# Autodesk Inventor assembly: Draft_02_Combined
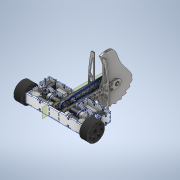
[picture p0: Inventor's stored thumbnail of the model, 180x180]
Saved by Autodesk Inventor 2022 (Build 260153000, 153)
## iProperties
Created: 2021-03-10
Part Number: Draft_02_Combined
Document SubType Name: Assembly
Designer: M3rob
Mass: 100397 g
Surface Area: 45638.5 cm^2
Volume: 29165.9 cm^3
Density: 3.44228 g/cm^3
Author: M3rob
## Documents named in this file (33)
- C:\Users\M3rob\Documents\GrabCAD\FireBird 250 Pound Gaming Machine\Drafts\FrameDrafts\Draft_03\Draft_03_Combined.iam
- C:\Users\M3rob\Documents\GrabCAD\FireBird 250 Pound Gaming Machine\Drafts\FrameDrafts\Draft_03\NeckFrame_03.ipt
- C:\Users\M3rob\Documents\GrabCAD\FireBird 250 Pound Gaming Machine\Drafts\FrameDrafts\Draft_03\FrontWallFrame_03.ipt
- C:\Users\M3rob\Documents\GrabCAD\FireBird 250 Pound Gaming Machine\Drafts\FrameDrafts\Draft_03\BackWallFrame_03.ipt
- C:\Users\M3rob\Documents\GrabCAD\FireBird 250 Pound Gaming Machine\Drafts\FrameDrafts\Draft_03\SmallSideFrame_03.ipt
- C:\Users\M3rob\Documents\GrabCAD\FireBird 250 Pound Gaming Machine\Drafts\FrameDrafts\Draft_03\DriveSideFrame_03.ipt
- C:\Users\M3rob\Documents\GrabCAD\FireBird 250 Pound Gaming Machine\Drafts\FrameDrafts\Draft_03\6524K421_FRICTION TORQUE LIMITER.ipt
- C:\Users\M3rob\Documents\GrabCAD\FireBird 250 Pound Gaming Machine\Drafts\FrameDrafts\Draft_03\MotorMountingPlates.ipt
- C:\Users\M3rob\Documents\GrabCAD\FireBird 250 Pound Gaming Machine\Drafts\FrameDrafts\Draft_03\MotorMockup.ipt
- C:\Users\M3rob\Documents\GrabCAD\FireBird 250 Pound Gaming Machine\Drafts\FrameDrafts\Draft_03\GearboxMockup.ipt
- C:\Users\M3rob\Documents\Inventor\Content Center Files\R2021\en-US\AS 2465(2)\AS 2465 - 3_8 x 1 1_4  UNC.ipt
- C:\Users\M3rob\Documents\Inventor\Content Center Files\R2021\en-US\AS 2465(1)\AS 2465 - 3_8  UNC(1).ipt
- C:\Users\M3rob\Documents\Inventor\Content Center Files\R2021\en-US\U UNC 2603(1)\Unbrako - 8 x 1 1_4 - 32 - 1.25 - Unbrako.ipt
- C:\Users\M3rob\Documents\Inventor\Content Center Files\R2021\en-US\U UNC 2603(1)\Unbrako - 5_16 x 1 3_4 - 18 - 1.75 - Unbrako.ipt
- C:\Users\M3rob\Documents\GrabCAD\FireBird 250 Pound Gaming Machine\Drafts\FrameDrafts\Draft_03\Chain Drive1.iam
- C:\Users\M3rob\Documents\GrabCAD\FireBird 250 Pound Gaming Machine\Drafts\FrameDrafts\Draft_03\Chain Drive2.iam
- C:\Users\M3rob\Documents\GrabCAD\FireBird 250 Pound Gaming Machine\Drafts\FrameDrafts\Draft_03\Chain Drive3.iam
- C:\Users\M3rob\Documents\GrabCAD\FireBird 250 Pound Gaming Machine\Drafts\FrameDrafts\Draft_03\Bearing1.iam
- C:\Users\M3rob\Documents\GrabCAD\FireBird 250 Pound Gaming Machine\Drafts\FrameDrafts\Draft_03\Shaft4.ipt
- C:\Users\M3rob\Documents\GrabCAD\FireBird 250 Pound Gaming Machine\Drafts\FrameDrafts\Draft_03\WeaponDraft02.ipt
- C:\Users\M3rob\Documents\GrabCAD\FireBird 250 Pound Gaming Machine\Drafts\FrameDrafts\Draft_03\Bearing3.iam
- C:\Users\M3rob\Documents\GrabCAD\FireBird 250 Pound Gaming Machine\Drafts\FrameDrafts\Draft_03\Shaft5.ipt
- C:\Users\M3rob\Documents\GrabCAD\FireBird 250 Pound Gaming Machine\Drafts\FrameDrafts\Draft_03\MotorCircularClamp.ipt
- C:\Users\M3rob\Documents\GrabCAD\FireBird 250 Pound Gaming Machine\Drafts\FrameDrafts\Draft_03\MotorClampUhmw.ipt
- C:\Users\M3rob\Documents\GrabCAD\FireBird 250 Pound Gaming Machine\Drafts\FrameDrafts\Draft_03\MockupWheel.ipt
- C:\Users\M3rob\Documents\GrabCAD\FireBird 250 Pound Gaming Machine\Drafts\FrameDrafts\Draft_03\WheelHubMockup.ipt
- C:\Users\M3rob\Documents\GrabCAD\FireBird 250 Pound Gaming Machine\Drafts\FrameDrafts\Draft_03\ThiccUpright.ipt
- C:\Users\M3rob\Documents\GrabCAD\FireBird 250 Pound Gaming Machine\Battery Mockup.ipt
- C:\Users\M3rob\Documents\GrabCAD\FireBird 250 Pound Gaming Machine\EscMockup.ipt
- C:\Users\M3rob\Documents\GrabCAD\FireBird 250 Pound Gaming Machine\Whyachi_MS-2PowerSwitch.ipt
- C:\Users\M3rob\Documents\GrabCAD\FireBird 250 Pound Gaming Machine\Drafts\FrameDrafts\Draft_03\AdaptiveTopPlate03.ipt
- C:\Users\M3rob\Documents\GrabCAD\FireBird 250 Pound Gaming Machine\Drafts\FrameDrafts\Draft_03\MidWallFrame_03.ipt
- C:\Users\M3rob\Documents\Inventor\Content Center Files\R2021\en-US\ANSI B18.2.2(06)\ANSI B18.2.2 - 3_8 - 16(06).ipt
## Components (147 placed, 28 different names)
1. NeckFrame_03:1 — Mate:1, Mate:3, Mate:4, Mate:5, Mate:12, Mate:14, Mate:17, Mate:18, Mate:40, Mate:41, Mate:42, Mate:47, Mate:71, Mate:73, Mate:75, Mate:77, Mate:98, Mate:99, Mate:104, Flush:4, Mate:125, Flush:18, Mate:260, Mate:384, Mate:385, Mate:386
2. NeckFrame_03:2 — Mate:1, Mate:6, Mate:7, Mate:8, Mate:9, Mate:10, Mate:11, Mate:19, Mate:43, Mate:44, Mate:45, Mate:46, Mate:87, Mate:89, Mate:91, Mate:93, Mate:103, Mate:105, Flush:3, Mate:110, Mate:111, Mate:123, Mate:124, Mate:381, Mate:382, Mate:383
3. MidWallFrame_03:1 — Mate:9, Mate:10, Mate:11, Mate:20, Mate:21, Mate:22, Mate:32, Mate:33, Mate:34, Mate:405, Mate:437, Mate:439
4. FrontWallFrame_03:2 — Mate:6, Mate:7, Mate:8, Flush:41, Flush:50, Mate:433, Mate:434, Mate:483, Mate:485, Mate:487, Mate:489, Mate:491, Mate:493, Mate:495, Mate:497, Mate:499, Mate:501, Mate:503, Mate:505, Mate:507, Mate:509
5. FrontWallFrame_03:3 — Mate:3, Mate:4, Mate:5, Mate:23, Mate:24, Mate:25, Mate:442, Mate:445, Flush:53, Mate:447, Mate:448, Mate:539, Mate:541, Mate:543, Mate:545, Mate:547, Mate:549, Mate:551, Mate:553, Mate:555, Mate:557, Mate:559, Mate:561, Mate:563, Mate:565
6. MidWallFrame_03:2 — Mate:12, Mate:14, Mate:39, Mate:260, Mate:410, Mate:451
7. BackWallFrame_03:1 — Mate:17, Mate:18, Mate:19, Mate:35, Mate:37, Mate:38
8. SmallSideFrame_03:1 — Mate:20, Mate:21, Mate:22, Flush:42, Mate:436
9. SmallSideFrame_03:2 — Mate:23, Mate:24, Mate:25, Mate:440
10. DriveSideFrame_03:1 — Mate:32, Mate:33, Mate:34, Mate:35, Insert:9, Insert:10, Insert:11, Insert:12, Mate:378, Mate:379, Mate:380, Insert:27, Mate:411, Mate:438, Flush:52
11. DriveSideFrame_03:2 — Mate:37, Mate:38, Mate:39, Mate:57, Mate:59, Insert:13, Insert:14, Insert:15, Insert:16, Mate:377, Insert:29, Flush:40, Mate:450, Flush:54
12. 6524K421_FRICTION TORQUE LIMITER:1 — Mate:94, Flush:2, Mate:96
13. 6524K421_FRICTION TORQUE LIMITER:2 — Mate:95, Flush:1, Mate:97
14. Chain Drive:1 [sub-assembly]
15. Chain Drive:2 [sub-assembly] — Mate:112, Mate:452
16. Chain Drive:3 [sub-assembly]
17. Bearing:1 [sub-assembly] — Mate:103, Mate:104
18. Bearing:2 [sub-assembly] — Mate:105, Flush:3
19. Shaft:1 — Mate:112, Mate:113, Angle:1
20. WeaponDraft02:1 — Mate:110, Mate:111
21. Bearing:3 [sub-assembly] — Mate:123, Mate:124
22. ThiccUpright:1 — Mate:381, Mate:382, Mate:383
23. ThiccUpright:2 — Mate:384, Mate:385, Mate:386
24. AdaptiveTopPlate03 — Flush:40, Mate:454, Mate:455, Mate:456, Mate:457, Mate:458, Mate:459, Mate:460, Mate:461, Mate:462, Mate:463, Mate:464, Mate:465, Mate:466, Mate:467, Mate:468, Mate:469, Mate:470, Mate:471, Mate:472, Mate:473, Mate:474, Mate:475, Mate:476, Mate:477, Mate:478, Mate:479, Mate:480, Mate:481, Mate:482, Mate:484, Mate:486, Mate:488, Mate:490, Mate:492, Mate:494, Mate:496, Mate:498, Mate:500, Mate:502, Mate:504, Mate:506, Mate:508
25. AdaptiveTopPlate03:2 — Mate:411, Flush:41, Flush:42, Mate:421, Mate:422, Mate:441, Mate:444, Mate:446, Mate:510, Mate:511, Mate:512, Mate:513, Mate:514, Mate:515, Mate:516, Mate:517, Mate:518, Mate:519, Mate:520, Mate:521, Mate:522, Mate:523, Mate:524, Mate:525, Mate:526, Mate:527, Mate:528, Mate:529, Mate:530, Mate:531, Mate:532, Mate:533, Mate:534, Mate:535, Mate:536, Mate:537, Mate:538, Mate:540, Mate:542, Mate:544, Mate:546, Mate:548, Mate:550, Mate:552, Mate:554, Mate:556, Mate:558, Mate:560, Mate:562, Mate:564
26. Whyachi_MS-2PowerSwitch:3 — Mate:438, Mate:439, Flush:52
27. SmallSideFrame_03:3 — Flush:50, Mate:433, Mate:434, Mate:435
28. EscMockup:5 — Mate:443, Mate:444, Mate:445
29. SmallSideFrame_03:4 — Flush:53, Mate:447, Mate:448, Mate:449
30. AS 2465 - Inch 3/8 x 1 1/4  UNC:9 — Mate:454, Mate:455
31. Hex Machine Screw Nut - Inch 3/8 - 16:1 — Mate:482, Mate:483
32. AS 2465 - Inch 3/8 x 1 1/4  UNC:10 — Mate:456, Mate:457
33. AS 2465 - Inch 3/8 x 1 1/4  UNC:11 — Mate:458, Mate:459
34. AS 2465 - Inch 3/8 x 1 1/4  UNC:12 — Mate:460, Mate:461
35. AS 2465 - Inch 3/8 x 1 1/4  UNC:13 — Mate:462, Mate:463
36. AS 2465 - Inch 3/8 x 1 1/4  UNC:14 — Mate:464, Mate:465
37. AS 2465 - Inch 3/8 x 1 1/4  UNC:15 — Mate:466, Mate:467
38. AS 2465 - Inch 3/8 x 1 1/4  UNC:16 — Mate:468, Mate:469
39. AS 2465 - Inch 3/8 x 1 1/4  UNC:17 — Mate:470, Mate:471
40. AS 2465 - Inch 3/8 x 1 1/4  UNC:18 — Mate:472, Mate:473
41. AS 2465 - Inch 3/8 x 1 1/4  UNC:19 — Mate:474, Mate:475
42. AS 2465 - Inch 3/8 x 1 1/4  UNC:20 — Mate:476, Mate:477
43. AS 2465 - Inch 3/8 x 1 1/4  UNC:21 — Mate:478, Mate:479
44. AS 2465 - Inch 3/8 x 1 1/4  UNC:22 — Mate:480, Mate:481
45. Hex Machine Screw Nut - Inch 3/8 - 16:2 — Mate:484, Mate:485
46. Hex Machine Screw Nut - Inch 3/8 - 16:3 — Mate:486, Mate:487
47. Hex Machine Screw Nut - Inch 3/8 - 16:4 — Mate:488, Mate:489
48. Hex Machine Screw Nut - Inch 3/8 - 16:5 — Mate:490, Mate:491
49. Hex Machine Screw Nut - Inch 3/8 - 16:6 — Mate:492, Mate:493
50. Hex Machine Screw Nut - Inch 3/8 - 16:7 — Mate:494, Mate:495
51. Hex Machine Screw Nut - Inch 3/8 - 16:8 — Mate:496, Mate:497
52. Hex Machine Screw Nut - Inch 3/8 - 16:9 — Mate:498, Mate:499
53. Hex Machine Screw Nut - Inch 3/8 - 16:10 — Mate:500, Mate:501
54. Hex Machine Screw Nut - Inch 3/8 - 16:11 — Mate:502, Mate:503
55. Hex Machine Screw Nut - Inch 3/8 - 16:12 — Mate:504, Mate:505
56. Hex Machine Screw Nut - Inch 3/8 - 16:13 — Mate:506, Mate:507
57. Hex Machine Screw Nut - Inch 3/8 - 16:14 — Mate:508, Mate:509
58. AS 2465 - Inch 3/8 x 1 1/4  UNC:23 — Mate:510, Mate:511
59. Hex Machine Screw Nut - Inch 3/8 - 16:15 — Mate:538, Mate:539
60. AS 2465 - Inch 3/8 x 1 1/4  UNC:24 — Mate:512, Mate:513
61. AS 2465 - Inch 3/8 x 1 1/4  UNC:25 — Mate:514, Mate:515
62. AS 2465 - Inch 3/8 x 1 1/4  UNC:26 — Mate:516, Mate:517
63. AS 2465 - Inch 3/8 x 1 1/4  UNC:27 — Mate:518, Mate:519
64. AS 2465 - Inch 3/8 x 1 1/4  UNC:28 — Mate:520, Mate:521
65. AS 2465 - Inch 3/8 x 1 1/4  UNC:29 — Mate:522, Mate:523
66. AS 2465 - Inch 3/8 x 1 1/4  UNC:30 — Mate:524, Mate:525
67. AS 2465 - Inch 3/8 x 1 1/4  UNC:31 — Mate:526, Mate:527
68. AS 2465 - Inch 3/8 x 1 1/4  UNC:32 — Mate:528, Mate:529
69. AS 2465 - Inch 3/8 x 1 1/4  UNC:33 — Mate:530, Mate:531
70. AS 2465 - Inch 3/8 x 1 1/4  UNC:34 — Mate:532, Mate:533
71. AS 2465 - Inch 3/8 x 1 1/4  UNC:35 — Mate:534, Mate:535
72. AS 2465 - Inch 3/8 x 1 1/4  UNC:36 — Mate:536, Mate:537
73. Hex Machine Screw Nut - Inch 3/8 - 16:16 — Mate:540, Mate:541
74. Hex Machine Screw Nut - Inch 3/8 - 16:17 — Mate:542, Mate:543
75. Hex Machine Screw Nut - Inch 3/8 - 16:18 — Mate:544, Mate:545
76. Hex Machine Screw Nut - Inch 3/8 - 16:19 — Mate:546, Mate:547
77. Hex Machine Screw Nut - Inch 3/8 - 16:20 — Mate:548, Mate:549
78. Hex Machine Screw Nut - Inch 3/8 - 16:21 — Mate:550, Mate:551
79. Hex Machine Screw Nut - Inch 3/8 - 16:22 — Mate:552, Mate:553
80. Hex Machine Screw Nut - Inch 3/8 - 16:23 — Mate:554, Mate:555
81. Hex Machine Screw Nut - Inch 3/8 - 16:24 — Mate:556, Mate:557
82. Hex Machine Screw Nut - Inch 3/8 - 16:25 — Mate:558, Mate:559
83. Hex Machine Screw Nut - Inch 3/8 - 16:26 — Mate:560, Mate:561
84. Hex Machine Screw Nut - Inch 3/8 - 16:27 — Mate:562, Mate:563
85. Hex Machine Screw Nut - Inch 3/8 - 16:28 — Mate:564, Mate:565
86. MotorMountingPlates:1 — Mate:40, Mate:41, Mate:42, Mate:49, Mate:62, Mate:63, Mate:64, Mate:65, Mate:66, Mate:67, Mate:68, Mate:69, Mate:70, Mate:72, Mate:74, Mate:76, Insert:5, Insert:6, Insert:7, Insert:8, Mate:96
87. MotorMountingPlates:2 — Mate:43, Mate:44, Mate:45, Mate:50, Mate:78, Mate:79, Mate:80, Mate:81, Mate:82, Mate:83, Mate:84, Mate:85, Mate:86, Mate:88, Mate:90, Mate:92, Insert:1, Insert:2, Insert:3, Insert:4, Mate:97
88. MotorMockup:1 — Mate:46, Mate:50, Mate:95, Flush:1, Insert:21
89. MotorMockup:2 — Mate:47, Mate:49, Mate:94, Flush:2, Insert:24
90. MotorMockup:3 — Mate:60, Mate:61, Insert:23
91. MotorMockup:4 — Insert:22, Insert:25
92. GearboxMockup:1 — Mate:57, Mate:59, Mate:60, Mate:61, Mate:377, Angle:4
93. GearboxMockup:2 — Mate:378, Mate:379, Mate:380, Insert:25, Angle:3
94. AS 2465 - Inch 3/8 x 1 1/4  UNC:1 — Mate:62, Mate:63
95. AS 2465 - Inch 3/8  UNC:1 — Mate:70, Mate:71
96. AS 2465 - Inch 3/8 x 1 1/4  UNC:2 — Mate:64, Mate:65
97. AS 2465 - Inch 3/8 x 1 1/4  UNC:3 — Mate:66, Mate:67
98. AS 2465 - Inch 3/8 x 1 1/4  UNC:4 — Mate:68, Mate:69
99. AS 2465 - Inch 3/8  UNC:2 — Mate:72, Mate:73
100. AS 2465 - Inch 3/8  UNC:3 — Mate:74, Mate:75
101. AS 2465 - Inch 3/8  UNC:4 — Mate:76, Mate:77
102. AS 2465 - Inch 3/8 x 1 1/4  UNC:5 — Mate:78, Mate:79
103. AS 2465 - Inch 3/8  UNC:5 — Mate:86, Mate:87
104. AS 2465 - Inch 3/8 x 1 1/4  UNC:6 — Mate:80, Mate:81
105. AS 2465 - Inch 3/8 x 1 1/4  UNC:7 — Mate:82, Mate:83
106. AS 2465 - Inch 3/8 x 1 1/4  UNC:8 — Mate:84, Mate:85
107. AS 2465 - Inch 3/8  UNC:6 — Mate:88, Mate:89
108. AS 2465 - Inch 3/8  UNC:7 — Mate:90, Mate:91
109. AS 2465 - Inch 3/8  UNC:8 — Mate:92, Mate:93
110. Unbrako UNC Hex Socket Cap - Inch 8 x 1 1/4:1 — Insert:1
111. Unbrako UNC Hex Socket Cap - Inch 8 x 1 1/4:2 — Insert:2
112. Unbrako UNC Hex Socket Cap - Inch 8 x 1 1/4:3 — Insert:3
113. Unbrako UNC Hex Socket Cap - Inch 8 x 1 1/4:4 — Insert:4
114. Unbrako UNC Hex Socket Cap - Inch 8 x 1 1/4:5 — Insert:5
115. Unbrako UNC Hex Socket Cap - Inch 8 x 1 1/4:6 — Insert:6
116. Unbrako UNC Hex Socket Cap - Inch 8 x 1 1/4:7 — Insert:7
117. Unbrako UNC Hex Socket Cap - Inch 8 x 1 1/4:8 — Insert:8
118. Unbrako UNC Hex Socket Cap - Inch 5/16 x 1 3/4:1 — Insert:9
119. Unbrako UNC Hex Socket Cap - Inch 5/16 x 1 3/4:2 — Insert:10
120. Unbrako UNC Hex Socket Cap - Inch 5/16 x 1 3/4:3 — Insert:11
121. Unbrako UNC Hex Socket Cap - Inch 5/16 x 1 3/4:4 — Insert:12
122. Unbrako UNC Hex Socket Cap - Inch 5/16 x 1 3/4:5 — Insert:13
123. Unbrako UNC Hex Socket Cap - Inch 5/16 x 1 3/4:6 — Insert:14
124. Unbrako UNC Hex Socket Cap - Inch 5/16 x 1 3/4:7 — Insert:15
125. Unbrako UNC Hex Socket Cap - Inch 5/16 x 1 3/4:8 — Insert:16
126. Bearing:4 [sub-assembly] — Mate:125, Flush:18
127. Shaft:1 — Mate:452, Mate:453, Angle:5
128. MockupWheel:1 — Insert:26
129. MockupWheel:2 — Insert:28
130. WheelHubMockup:1 — Insert:28, Insert:29, Angle:4
131. WheelHubMockup:2 — Insert:26, Insert:27, Angle:3
132. Whyachi_MS-2PowerSwitch:2 — Mate:450, Mate:451, Flush:54
133. EscMockup:1 — Mate:420, Mate:421, Flush:45, Flush:51
134. EscMockup:2 — Mate:420, Flush:45, Mate:436, Flush:51, Mate:437
135. EscMockup:4 — Mate:440, Mate:441, Mate:442, Mate:443
136. Battery Mockup:1 — Flush:28, Flush:32, Mate:405, Mate:424
137. Battery Mockup:2 — Flush:28, Flush:32, Mate:422, Mate:424, Mate:435
138. Battery Mockup:4 — Mate:388, Flush:24, Flush:31, Mate:410
139. Battery Mockup:5 — Mate:388, Flush:24, Flush:31, Mate:446, Mate:449
140. MotorCircularClamp:1 — Insert:19
141. MotorClampUhmw:1 — Insert:19, Insert:22
142. MotorCircularClamp:2 — Insert:20
143. MotorClampUhmw:2 — Insert:20, Insert:21
144. MotorCircularClamp:3 — Insert:18
145. MotorClampUhmw:3 — Insert:18, Insert:24
146. MotorCircularClamp:4 — Insert:17
147. MotorClampUhmw:4 — Insert:17, Insert:23
## Relationships (297: Mate 246, Insert 29, Flush 18, Angle 4)
- Mate:1: NeckFrame_03:1 ↔ NeckFrame_03:2
- Mate:3: NeckFrame_03:1 ↔ FrontWallFrame_03:3
- Mate:4: NeckFrame_03:1 ↔ FrontWallFrame_03:3
- Mate:5: NeckFrame_03:1 ↔ FrontWallFrame_03:3
- Mate:6: NeckFrame_03:2 ↔ FrontWallFrame_03:2
- Mate:7: NeckFrame_03:2 ↔ FrontWallFrame_03:2
- Mate:8: NeckFrame_03:2 ↔ FrontWallFrame_03:2
- Mate:9: NeckFrame_03:2 ↔ MidWallFrame_03:1
- Mate:10: NeckFrame_03:2 ↔ MidWallFrame_03:1
- Mate:11: NeckFrame_03:2 ↔ MidWallFrame_03:1
- Mate:12: NeckFrame_03:1 ↔ MidWallFrame_03:2
- Mate:14: NeckFrame_03:1 ↔ MidWallFrame_03:2
- Mate:17: NeckFrame_03:1 ↔ BackWallFrame_03:1
- Mate:18: NeckFrame_03:1 ↔ BackWallFrame_03:1
- Mate:19: NeckFrame_03:2 ↔ BackWallFrame_03:1
- Mate:20: MidWallFrame_03:1 ↔ SmallSideFrame_03:1
- Mate:21: MidWallFrame_03:1 ↔ SmallSideFrame_03:1
- Mate:22: MidWallFrame_03:1 ↔ SmallSideFrame_03:1
- Mate:23: FrontWallFrame_03:3 ↔ SmallSideFrame_03:2
- Mate:24: FrontWallFrame_03:3 ↔ SmallSideFrame_03:2
- Mate:25: FrontWallFrame_03:3 ↔ SmallSideFrame_03:2
- Mate:32: MidWallFrame_03:1 ↔ DriveSideFrame_03:1
- Mate:33: MidWallFrame_03:1 ↔ DriveSideFrame_03:1
- Mate:34: MidWallFrame_03:1 ↔ DriveSideFrame_03:1
- Mate:35: BackWallFrame_03:1 ↔ DriveSideFrame_03:1
- Mate:37: BackWallFrame_03:1 ↔ DriveSideFrame_03:2
- Mate:38: BackWallFrame_03:1 ↔ DriveSideFrame_03:2
- Mate:39: MidWallFrame_03:2 ↔ DriveSideFrame_03:2
- Mate:40: NeckFrame_03:1 ↔ MotorMountingPlates:1
- Mate:41: NeckFrame_03:1 ↔ MotorMountingPlates:1
- Mate:42: NeckFrame_03:1 ↔ MotorMountingPlates:1
- Mate:43: NeckFrame_03:2 ↔ MotorMountingPlates:2
- Mate:44: NeckFrame_03:2 ↔ MotorMountingPlates:2
- Mate:45: NeckFrame_03:2 ↔ MotorMountingPlates:2
- Mate:46: NeckFrame_03:2 ↔ MotorMockup:1
- Mate:47: NeckFrame_03:1 ↔ MotorMockup:2
- Mate:49: MotorMountingPlates:1 ↔ MotorMockup:2
- Mate:50: MotorMountingPlates:2 ↔ MotorMockup:1
- Mate:57: DriveSideFrame_03:2 ↔ GearboxMockup:1
- Mate:59: DriveSideFrame_03:2 ↔ GearboxMockup:1
- Mate:60: MotorMockup:3 ↔ GearboxMockup:1
- Mate:61: MotorMockup:3 ↔ GearboxMockup:1
- Mate:62: MotorMountingPlates:1 ↔ AS 2465 - Inch 3/8 x 1 1/4  UNC:1
- Mate:63: MotorMountingPlates:1 ↔ AS 2465 - Inch 3/8 x 1 1/4  UNC:1
- Mate:64: MotorMountingPlates:1 ↔ AS 2465 - Inch 3/8 x 1 1/4  UNC:2
- Mate:65: MotorMountingPlates:1 ↔ AS 2465 - Inch 3/8 x 1 1/4  UNC:2
- Mate:66: MotorMountingPlates:1 ↔ AS 2465 - Inch 3/8 x 1 1/4  UNC:3
- Mate:67: MotorMountingPlates:1 ↔ AS 2465 - Inch 3/8 x 1 1/4  UNC:3
- Mate:68: MotorMountingPlates:1 ↔ AS 2465 - Inch 3/8 x 1 1/4  UNC:4
- Mate:69: MotorMountingPlates:1 ↔ AS 2465 - Inch 3/8 x 1 1/4  UNC:4
- Mate:70: MotorMountingPlates:1 ↔ AS 2465 - Inch 3/8  UNC:1
- Mate:71: NeckFrame_03:1 ↔ AS 2465 - Inch 3/8  UNC:1
- Mate:72: MotorMountingPlates:1 ↔ AS 2465 - Inch 3/8  UNC:2
- Mate:73: NeckFrame_03:1 ↔ AS 2465 - Inch 3/8  UNC:2
- Mate:74: MotorMountingPlates:1 ↔ AS 2465 - Inch 3/8  UNC:3
- Mate:75: NeckFrame_03:1 ↔ AS 2465 - Inch 3/8  UNC:3
- Mate:76: MotorMountingPlates:1 ↔ AS 2465 - Inch 3/8  UNC:4
- Mate:77: NeckFrame_03:1 ↔ AS 2465 - Inch 3/8  UNC:4
- Mate:78: MotorMountingPlates:2 ↔ AS 2465 - Inch 3/8 x 1 1/4  UNC:5
- Mate:79: MotorMountingPlates:2 ↔ AS 2465 - Inch 3/8 x 1 1/4  UNC:5
- Mate:80: MotorMountingPlates:2 ↔ AS 2465 - Inch 3/8 x 1 1/4  UNC:6
- Mate:81: MotorMountingPlates:2 ↔ AS 2465 - Inch 3/8 x 1 1/4  UNC:6
- Mate:82: MotorMountingPlates:2 ↔ AS 2465 - Inch 3/8 x 1 1/4  UNC:7
- Mate:83: MotorMountingPlates:2 ↔ AS 2465 - Inch 3/8 x 1 1/4  UNC:7
- Mate:84: MotorMountingPlates:2 ↔ AS 2465 - Inch 3/8 x 1 1/4  UNC:8
- Mate:85: MotorMountingPlates:2 ↔ AS 2465 - Inch 3/8 x 1 1/4  UNC:8
- Mate:86: MotorMountingPlates:2 ↔ AS 2465 - Inch 3/8  UNC:5
- Mate:87: NeckFrame_03:2 ↔ AS 2465 - Inch 3/8  UNC:5
- Mate:88: MotorMountingPlates:2 ↔ AS 2465 - Inch 3/8  UNC:6
- Mate:89: NeckFrame_03:2 ↔ AS 2465 - Inch 3/8  UNC:6
- Mate:90: MotorMountingPlates:2 ↔ AS 2465 - Inch 3/8  UNC:7
- Mate:91: NeckFrame_03:2 ↔ AS 2465 - Inch 3/8  UNC:7
- Mate:92: MotorMountingPlates:2 ↔ AS 2465 - Inch 3/8  UNC:8
- Mate:93: NeckFrame_03:2 ↔ AS 2465 - Inch 3/8  UNC:8
- Insert:1: MotorMountingPlates:2 ↔ Unbrako UNC Hex Socket Cap - Inch 8 x 1 1/4:1
- Insert:2: MotorMountingPlates:2 ↔ Unbrako UNC Hex Socket Cap - Inch 8 x 1 1/4:2
- Insert:3: MotorMountingPlates:2 ↔ Unbrako UNC Hex Socket Cap - Inch 8 x 1 1/4:3
- Insert:4: MotorMountingPlates:2 ↔ Unbrako UNC Hex Socket Cap - Inch 8 x 1 1/4:4
- Insert:5: MotorMountingPlates:1 ↔ Unbrako UNC Hex Socket Cap - Inch 8 x 1 1/4:5
- Insert:6: MotorMountingPlates:1 ↔ Unbrako UNC Hex Socket Cap - Inch 8 x 1 1/4:6
- Insert:7: MotorMountingPlates:1 ↔ Unbrako UNC Hex Socket Cap - Inch 8 x 1 1/4:7
- Insert:8: MotorMountingPlates:1 ↔ Unbrako UNC Hex Socket Cap - Inch 8 x 1 1/4:8
- Insert:9: DriveSideFrame_03:1 ↔ Unbrako UNC Hex Socket Cap - Inch 5/16 x 1 3/4:1
- Insert:10: DriveSideFrame_03:1 ↔ Unbrako UNC Hex Socket Cap - Inch 5/16 x 1 3/4:2
- Insert:11: DriveSideFrame_03:1 ↔ Unbrako UNC Hex Socket Cap - Inch 5/16 x 1 3/4:3
- Insert:12: DriveSideFrame_03:1 ↔ Unbrako UNC Hex Socket Cap - Inch 5/16 x 1 3/4:4
- Insert:13: DriveSideFrame_03:2 ↔ Unbrako UNC Hex Socket Cap - Inch 5/16 x 1 3/4:5
- Insert:14: DriveSideFrame_03:2 ↔ Unbrako UNC Hex Socket Cap - Inch 5/16 x 1 3/4:6
- Insert:15: DriveSideFrame_03:2 ↔ Unbrako UNC Hex Socket Cap - Inch 5/16 x 1 3/4:7
- Insert:16: DriveSideFrame_03:2 ↔ Unbrako UNC Hex Socket Cap - Inch 5/16 x 1 3/4:8
- Mate:94: 6524K421_FRICTION TORQUE LIMITER:1 ↔ MotorMockup:2
- Mate:95: 6524K421_FRICTION TORQUE LIMITER:2 ↔ MotorMockup:1
- Flush:1: 6524K421_FRICTION TORQUE LIMITER:2 ↔ MotorMockup:1
- Flush:2: 6524K421_FRICTION TORQUE LIMITER:1 ↔ MotorMockup:2
- Mate:96 (1.5875 mm): 6524K421_FRICTION TORQUE LIMITER:1 ↔ MotorMountingPlates:1
- Mate:97 (1.5875 mm): 6524K421_FRICTION TORQUE LIMITER:2 ↔ MotorMountingPlates:2
- Mate:98: NeckFrame_03:1
- Mate:99: NeckFrame_03:1
- Mate:100
- Mate:101
- Mate:103: NeckFrame_03:2 ↔ Bearing:1
- Mate:104: NeckFrame_03:1 ↔ Bearing:1
- Mate:105: NeckFrame_03:2 ↔ Bearing:2
- Flush:3: NeckFrame_03:2 ↔ Bearing:2
- Flush:4 (19.05 mm): NeckFrame_03:1
- Mate:108
- Mate:109
- Mate:110: NeckFrame_03:2 ↔ WeaponDraft02:1
- Mate:111 (25.4 mm): NeckFrame_03:2 ↔ WeaponDraft02:1
- Mate:112: Chain Drive:2 ↔ Shaft:1
- Mate:113: Shaft:1
- Angle:1 (0 deg): Shaft:1
- Mate:123: NeckFrame_03:2 ↔ Bearing:3
- Mate:124: NeckFrame_03:2 ↔ Bearing:3
- Mate:125: NeckFrame_03:1 ↔ Bearing:4
- Flush:18: NeckFrame_03:1 ↔ Bearing:4
- Mate:260: NeckFrame_03:1 ↔ MidWallFrame_03:2
- Insert:17: MotorCircularClamp:4 ↔ MotorClampUhmw:4
- Insert:18: MotorCircularClamp:3 ↔ MotorClampUhmw:3
- Insert:19: MotorCircularClamp:1 ↔ MotorClampUhmw:1
- Insert:20: MotorCircularClamp:2 ↔ MotorClampUhmw:2
- Insert:21 (12.7 mm): MotorMockup:1 ↔ MotorClampUhmw:2
- Insert:22 (12.7 mm): MotorMockup:4 ↔ MotorClampUhmw:1
- Insert:23 (12.7 mm): MotorMockup:3 ↔ MotorClampUhmw:4
- Insert:24 (12.7 mm): MotorMockup:2 ↔ MotorClampUhmw:3
- Mate:377: DriveSideFrame_03:2 ↔ GearboxMockup:1
- Mate:378: DriveSideFrame_03:1 ↔ GearboxMockup:2
- Mate:379: DriveSideFrame_03:1 ↔ GearboxMockup:2
- Mate:380: DriveSideFrame_03:1 ↔ GearboxMockup:2
- Insert:25: MotorMockup:4 ↔ GearboxMockup:2
- Mate:381: NeckFrame_03:2 ↔ ThiccUpright:1
- Mate:382: NeckFrame_03:2 ↔ ThiccUpright:1
- Mate:383: NeckFrame_03:2 ↔ ThiccUpright:1
- Mate:384: NeckFrame_03:1 ↔ ThiccUpright:2
- Mate:385: NeckFrame_03:1 ↔ ThiccUpright:2
- Mate:386: NeckFrame_03:1 ↔ ThiccUpright:2
- Mate:388: Battery Mockup:4 ↔ Battery Mockup:5
- Flush:24: Battery Mockup:4 ↔ Battery Mockup:5
- Flush:28: Battery Mockup:1 ↔ Battery Mockup:2
- Flush:31: Battery Mockup:4 ↔ Battery Mockup:5
- Insert:26 (-6.35 mm): MockupWheel:1 ↔ WheelHubMockup:2
- Insert:27: DriveSideFrame_03:1 ↔ WheelHubMockup:2
- Angle:3 (0 deg): GearboxMockup:2 ↔ WheelHubMockup:2
- Insert:28 (-6.35 mm): MockupWheel:2 ↔ WheelHubMockup:1
- Insert:29: DriveSideFrame_03:2 ↔ WheelHubMockup:1
- Angle:4 (0 deg): GearboxMockup:1 ↔ WheelHubMockup:1
- Flush:32: Battery Mockup:1 ↔ Battery Mockup:2
- Mate:405 (3.175 mm): MidWallFrame_03:1 ↔ Battery Mockup:1
- Mate:410: MidWallFrame_03:2 ↔ Battery Mockup:4
- Flush:40: DriveSideFrame_03:2 ↔ AdaptiveTopPlate03
- Mate:411: DriveSideFrame_03:1 ↔ AdaptiveTopPlate03:2
- Flush:41: FrontWallFrame_03:2 ↔ AdaptiveTopPlate03:2
- Flush:42: SmallSideFrame_03:1 ↔ AdaptiveTopPlate03:2
- Mate:420 (6.35 mm): EscMockup:1 ↔ EscMockup:2
- Mate:421 (6.35 mm): AdaptiveTopPlate03:2 ↔ EscMockup:1
- Mate:422: AdaptiveTopPlate03:2 ↔ Battery Mockup:2
- Mate:424: Battery Mockup:1 ↔ Battery Mockup:2
- Flush:45: EscMockup:1 ↔ EscMockup:2
- Flush:50: FrontWallFrame_03:2 ↔ SmallSideFrame_03:3
- Mate:433: FrontWallFrame_03:2 ↔ SmallSideFrame_03:3
- Mate:434: FrontWallFrame_03:2 ↔ SmallSideFrame_03:3
- Mate:435 (6.35 mm): SmallSideFrame_03:3 ↔ Battery Mockup:2
- Mate:436 (6.35 mm): SmallSideFrame_03:1 ↔ EscMockup:2
- Flush:51: EscMockup:1 ↔ EscMockup:2
- Mate:437 (6.35 mm): MidWallFrame_03:1 ↔ EscMockup:2
- Mate:438: DriveSideFrame_03:1 ↔ Whyachi_MS-2PowerSwitch:3
- Mate:439: MidWallFrame_03:1 ↔ Whyachi_MS-2PowerSwitch:3
- Flush:52: DriveSideFrame_03:1 ↔ Whyachi_MS-2PowerSwitch:3
- Mate:440 (6.35 mm): SmallSideFrame_03:2 ↔ EscMockup:4
- Mate:441 (6.35 mm): AdaptiveTopPlate03:2 ↔ EscMockup:4
- Mate:442 (6.35 mm): FrontWallFrame_03:3 ↔ EscMockup:4
- Mate:443 (6.35 mm): EscMockup:5 ↔ EscMockup:4
- Mate:444 (6.35 mm): AdaptiveTopPlate03:2 ↔ EscMockup:5
- Mate:445 (6.35 mm): FrontWallFrame_03:3 ↔ EscMockup:5
- Mate:446 (6.35 mm): AdaptiveTopPlate03:2 ↔ Battery Mockup:5
- Flush:53: FrontWallFrame_03:3 ↔ SmallSideFrame_03:4
- Mate:447: FrontWallFrame_03:3 ↔ SmallSideFrame_03:4
- Mate:448: FrontWallFrame_03:3 ↔ SmallSideFrame_03:4
- Mate:449 (6.35 mm): SmallSideFrame_03:4 ↔ Battery Mockup:5
- Mate:450: DriveSideFrame_03:2 ↔ Whyachi_MS-2PowerSwitch:2
- Mate:451: MidWallFrame_03:2 ↔ Whyachi_MS-2PowerSwitch:2
- Flush:54: DriveSideFrame_03:2 ↔ Whyachi_MS-2PowerSwitch:2
- Mate:452: Chain Drive:2 ↔ Shaft:1
- Mate:453: Shaft:1
- Angle:5 (0 deg): Shaft:1
- Mate:454: AdaptiveTopPlate03 ↔ AS 2465 - Inch 3/8 x 1 1/4  UNC:9
- Mate:455: AdaptiveTopPlate03 ↔ AS 2465 - Inch 3/8 x 1 1/4  UNC:9
- Mate:456: AdaptiveTopPlate03 ↔ AS 2465 - Inch 3/8 x 1 1/4  UNC:10
- Mate:457: AdaptiveTopPlate03 ↔ AS 2465 - Inch 3/8 x 1 1/4  UNC:10
- Mate:458: AdaptiveTopPlate03 ↔ AS 2465 - Inch 3/8 x 1 1/4  UNC:11
- Mate:459: AdaptiveTopPlate03 ↔ AS 2465 - Inch 3/8 x 1 1/4  UNC:11
- Mate:460: AdaptiveTopPlate03 ↔ AS 2465 - Inch 3/8 x 1 1/4  UNC:12
- Mate:461: AdaptiveTopPlate03 ↔ AS 2465 - Inch 3/8 x 1 1/4  UNC:12
- Mate:462: AdaptiveTopPlate03 ↔ AS 2465 - Inch 3/8 x 1 1/4  UNC:13
- Mate:463: AdaptiveTopPlate03 ↔ AS 2465 - Inch 3/8 x 1 1/4  UNC:13
- Mate:464: AdaptiveTopPlate03 ↔ AS 2465 - Inch 3/8 x 1 1/4  UNC:14
- Mate:465: AdaptiveTopPlate03 ↔ AS 2465 - Inch 3/8 x 1 1/4  UNC:14
- Mate:466: AdaptiveTopPlate03 ↔ AS 2465 - Inch 3/8 x 1 1/4  UNC:15
- Mate:467: AdaptiveTopPlate03 ↔ AS 2465 - Inch 3/8 x 1 1/4  UNC:15
- Mate:468: AdaptiveTopPlate03 ↔ AS 2465 - Inch 3/8 x 1 1/4  UNC:16
- Mate:469: AdaptiveTopPlate03 ↔ AS 2465 - Inch 3/8 x 1 1/4  UNC:16
- Mate:470: AdaptiveTopPlate03 ↔ AS 2465 - Inch 3/8 x 1 1/4  UNC:17
- Mate:471: AdaptiveTopPlate03 ↔ AS 2465 - Inch 3/8 x 1 1/4  UNC:17
- Mate:472: AdaptiveTopPlate03 ↔ AS 2465 - Inch 3/8 x 1 1/4  UNC:18
- Mate:473: AdaptiveTopPlate03 ↔ AS 2465 - Inch 3/8 x 1 1/4  UNC:18
- Mate:474: AdaptiveTopPlate03 ↔ AS 2465 - Inch 3/8 x 1 1/4  UNC:19
- Mate:475: AdaptiveTopPlate03 ↔ AS 2465 - Inch 3/8 x 1 1/4  UNC:19
- Mate:476: AdaptiveTopPlate03 ↔ AS 2465 - Inch 3/8 x 1 1/4  UNC:20
- Mate:477: AdaptiveTopPlate03 ↔ AS 2465 - Inch 3/8 x 1 1/4  UNC:20
- Mate:478: AdaptiveTopPlate03 ↔ AS 2465 - Inch 3/8 x 1 1/4  UNC:21
- Mate:479: AdaptiveTopPlate03 ↔ AS 2465 - Inch 3/8 x 1 1/4  UNC:21
- Mate:480: AdaptiveTopPlate03 ↔ AS 2465 - Inch 3/8 x 1 1/4  UNC:22
- Mate:481: AdaptiveTopPlate03 ↔ AS 2465 - Inch 3/8 x 1 1/4  UNC:22
- Mate:482: AdaptiveTopPlate03 ↔ Hex Machine Screw Nut - Inch 3/8 - 16:1
- Mate:483: FrontWallFrame_03:2 ↔ Hex Machine Screw Nut - Inch 3/8 - 16:1
- Mate:484: AdaptiveTopPlate03 ↔ Hex Machine Screw Nut - Inch 3/8 - 16:2
- Mate:485: FrontWallFrame_03:2 ↔ Hex Machine Screw Nut - Inch 3/8 - 16:2
- Mate:486: AdaptiveTopPlate03 ↔ Hex Machine Screw Nut - Inch 3/8 - 16:3
- Mate:487: FrontWallFrame_03:2 ↔ Hex Machine Screw Nut - Inch 3/8 - 16:3
- Mate:488: AdaptiveTopPlate03 ↔ Hex Machine Screw Nut - Inch 3/8 - 16:4
- Mate:489: FrontWallFrame_03:2 ↔ Hex Machine Screw Nut - Inch 3/8 - 16:4
- Mate:490: AdaptiveTopPlate03 ↔ Hex Machine Screw Nut - Inch 3/8 - 16:5
- Mate:491: FrontWallFrame_03:2 ↔ Hex Machine Screw Nut - Inch 3/8 - 16:5
- Mate:492: AdaptiveTopPlate03 ↔ Hex Machine Screw Nut - Inch 3/8 - 16:6
- Mate:493: FrontWallFrame_03:2 ↔ Hex Machine Screw Nut - Inch 3/8 - 16:6
- Mate:494: AdaptiveTopPlate03 ↔ Hex Machine Screw Nut - Inch 3/8 - 16:7
- Mate:495: FrontWallFrame_03:2 ↔ Hex Machine Screw Nut - Inch 3/8 - 16:7
- Mate:496: AdaptiveTopPlate03 ↔ Hex Machine Screw Nut - Inch 3/8 - 16:8
- Mate:497: FrontWallFrame_03:2 ↔ Hex Machine Screw Nut - Inch 3/8 - 16:8
- Mate:498: AdaptiveTopPlate03 ↔ Hex Machine Screw Nut - Inch 3/8 - 16:9
- Mate:499: FrontWallFrame_03:2 ↔ Hex Machine Screw Nut - Inch 3/8 - 16:9
- Mate:500: AdaptiveTopPlate03 ↔ Hex Machine Screw Nut - Inch 3/8 - 16:10
- Mate:501: FrontWallFrame_03:2 ↔ Hex Machine Screw Nut - Inch 3/8 - 16:10
- Mate:502: AdaptiveTopPlate03 ↔ Hex Machine Screw Nut - Inch 3/8 - 16:11
- Mate:503: FrontWallFrame_03:2 ↔ Hex Machine Screw Nut - Inch 3/8 - 16:11
- Mate:504: AdaptiveTopPlate03 ↔ Hex Machine Screw Nut - Inch 3/8 - 16:12
- Mate:505: FrontWallFrame_03:2 ↔ Hex Machine Screw Nut - Inch 3/8 - 16:12
- Mate:506: AdaptiveTopPlate03 ↔ Hex Machine Screw Nut - Inch 3/8 - 16:13
- Mate:507: FrontWallFrame_03:2 ↔ Hex Machine Screw Nut - Inch 3/8 - 16:13
- Mate:508: AdaptiveTopPlate03 ↔ Hex Machine Screw Nut - Inch 3/8 - 16:14
- Mate:509: FrontWallFrame_03:2 ↔ Hex Machine Screw Nut - Inch 3/8 - 16:14
- Mate:510: AdaptiveTopPlate03:2 ↔ AS 2465 - Inch 3/8 x 1 1/4  UNC:23
- Mate:511: AdaptiveTopPlate03:2 ↔ AS 2465 - Inch 3/8 x 1 1/4  UNC:23
- Mate:512: AdaptiveTopPlate03:2 ↔ AS 2465 - Inch 3/8 x 1 1/4  UNC:24
- Mate:513: AdaptiveTopPlate03:2 ↔ AS 2465 - Inch 3/8 x 1 1/4  UNC:24
- Mate:514: AdaptiveTopPlate03:2 ↔ AS 2465 - Inch 3/8 x 1 1/4  UNC:25
- Mate:515: AdaptiveTopPlate03:2 ↔ AS 2465 - Inch 3/8 x 1 1/4  UNC:25
- Mate:516: AdaptiveTopPlate03:2 ↔ AS 2465 - Inch 3/8 x 1 1/4  UNC:26
- Mate:517: AdaptiveTopPlate03:2 ↔ AS 2465 - Inch 3/8 x 1 1/4  UNC:26
- Mate:518: AdaptiveTopPlate03:2 ↔ AS 2465 - Inch 3/8 x 1 1/4  UNC:27
- Mate:519: AdaptiveTopPlate03:2 ↔ AS 2465 - Inch 3/8 x 1 1/4  UNC:27
- Mate:520: AdaptiveTopPlate03:2 ↔ AS 2465 - Inch 3/8 x 1 1/4  UNC:28
- Mate:521: AdaptiveTopPlate03:2 ↔ AS 2465 - Inch 3/8 x 1 1/4  UNC:28
- Mate:522: AdaptiveTopPlate03:2 ↔ AS 2465 - Inch 3/8 x 1 1/4  UNC:29
- Mate:523: AdaptiveTopPlate03:2 ↔ AS 2465 - Inch 3/8 x 1 1/4  UNC:29
- Mate:524: AdaptiveTopPlate03:2 ↔ AS 2465 - Inch 3/8 x 1 1/4  UNC:30
- Mate:525: AdaptiveTopPlate03:2 ↔ AS 2465 - Inch 3/8 x 1 1/4  UNC:30
- Mate:526: AdaptiveTopPlate03:2 ↔ AS 2465 - Inch 3/8 x 1 1/4  UNC:31
- Mate:527: AdaptiveTopPlate03:2 ↔ AS 2465 - Inch 3/8 x 1 1/4  UNC:31
- Mate:528: AdaptiveTopPlate03:2 ↔ AS 2465 - Inch 3/8 x 1 1/4  UNC:32
- Mate:529: AdaptiveTopPlate03:2 ↔ AS 2465 - Inch 3/8 x 1 1/4  UNC:32
- Mate:530: AdaptiveTopPlate03:2 ↔ AS 2465 - Inch 3/8 x 1 1/4  UNC:33
- Mate:531: AdaptiveTopPlate03:2 ↔ AS 2465 - Inch 3/8 x 1 1/4  UNC:33
- Mate:532: AdaptiveTopPlate03:2 ↔ AS 2465 - Inch 3/8 x 1 1/4  UNC:34
- Mate:533: AdaptiveTopPlate03:2 ↔ AS 2465 - Inch 3/8 x 1 1/4  UNC:34
- Mate:534: AdaptiveTopPlate03:2 ↔ AS 2465 - Inch 3/8 x 1 1/4  UNC:35
- Mate:535: AdaptiveTopPlate03:2 ↔ AS 2465 - Inch 3/8 x 1 1/4  UNC:35
- Mate:536: AdaptiveTopPlate03:2 ↔ AS 2465 - Inch 3/8 x 1 1/4  UNC:36
- Mate:537: AdaptiveTopPlate03:2 ↔ AS 2465 - Inch 3/8 x 1 1/4  UNC:36
- Mate:538: AdaptiveTopPlate03:2 ↔ Hex Machine Screw Nut - Inch 3/8 - 16:15
- Mate:539: FrontWallFrame_03:3 ↔ Hex Machine Screw Nut - Inch 3/8 - 16:15
- Mate:540: AdaptiveTopPlate03:2 ↔ Hex Machine Screw Nut - Inch 3/8 - 16:16
- Mate:541: FrontWallFrame_03:3 ↔ Hex Machine Screw Nut - Inch 3/8 - 16:16
- Mate:542: AdaptiveTopPlate03:2 ↔ Hex Machine Screw Nut - Inch 3/8 - 16:17
- Mate:543: FrontWallFrame_03:3 ↔ Hex Machine Screw Nut - Inch 3/8 - 16:17
- Mate:544: AdaptiveTopPlate03:2 ↔ Hex Machine Screw Nut - Inch 3/8 - 16:18
- Mate:545: FrontWallFrame_03:3 ↔ Hex Machine Screw Nut - Inch 3/8 - 16:18
- Mate:546: AdaptiveTopPlate03:2 ↔ Hex Machine Screw Nut - Inch 3/8 - 16:19
- Mate:547: FrontWallFrame_03:3 ↔ Hex Machine Screw Nut - Inch 3/8 - 16:19
- Mate:548: AdaptiveTopPlate03:2 ↔ Hex Machine Screw Nut - Inch 3/8 - 16:20
- Mate:549: FrontWallFrame_03:3 ↔ Hex Machine Screw Nut - Inch 3/8 - 16:20
- Mate:550: AdaptiveTopPlate03:2 ↔ Hex Machine Screw Nut - Inch 3/8 - 16:21
- Mate:551: FrontWallFrame_03:3 ↔ Hex Machine Screw Nut - Inch 3/8 - 16:21
- Mate:552: AdaptiveTopPlate03:2 ↔ Hex Machine Screw Nut - Inch 3/8 - 16:22
- Mate:553: FrontWallFrame_03:3 ↔ Hex Machine Screw Nut - Inch 3/8 - 16:22
- Mate:554: AdaptiveTopPlate03:2 ↔ Hex Machine Screw Nut - Inch 3/8 - 16:23
- Mate:555: FrontWallFrame_03:3 ↔ Hex Machine Screw Nut - Inch 3/8 - 16:23
- Mate:556: AdaptiveTopPlate03:2 ↔ Hex Machine Screw Nut - Inch 3/8 - 16:24
- Mate:557: FrontWallFrame_03:3 ↔ Hex Machine Screw Nut - Inch 3/8 - 16:24
- Mate:558: AdaptiveTopPlate03:2 ↔ Hex Machine Screw Nut - Inch 3/8 - 16:25
- Mate:559: FrontWallFrame_03:3 ↔ Hex Machine Screw Nut - Inch 3/8 - 16:25
- Mate:560: AdaptiveTopPlate03:2 ↔ Hex Machine Screw Nut - Inch 3/8 - 16:26
- Mate:561: FrontWallFrame_03:3 ↔ Hex Machine Screw Nut - Inch 3/8 - 16:26
- Mate:562: AdaptiveTopPlate03:2 ↔ Hex Machine Screw Nut - Inch 3/8 - 16:27
- Mate:563: FrontWallFrame_03:3 ↔ Hex Machine Screw Nut - Inch 3/8 - 16:27
- Mate:564: AdaptiveTopPlate03:2 ↔ Hex Machine Screw Nut - Inch 3/8 - 16:28
- Mate:565: FrontWallFrame_03:3 ↔ Hex Machine Screw Nut - Inch 3/8 - 16:28
